# Autodesk Inventor assembly: ASY MSC 202 LEFT BOARD
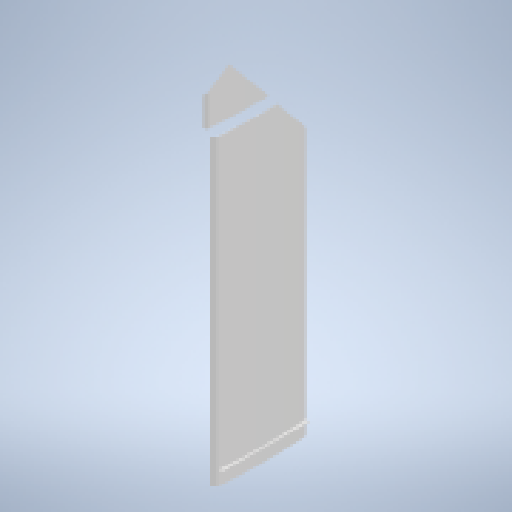
[picture p0: Inventor's stored thumbnail of the model, 512x512]
Saved by Autodesk Inventor 2025 (Build 290162010, 162A)
## iProperties
Created: 2024-07-21
Part Number: ASY MSC 202 LEFT BOARD
Document SubType Name: Assembly
Designer: pokla
Author: pokla
## Documents named in this file (6)
- C:\Users\admin\YandexDisk-badmisterfox\домашниий пк\Inventor\Manturovo\Manturovo_Se-clar\ASY MSC 202 LEFT BOARD.iam
- C:\Users\admin\YandexDisk-badmisterfox\домашниий пк\Inventor\Manturovo\Manturovo_Se-clar\MSC 052 rib board.ipt
- C:\Users\admin\YandexDisk-badmisterfox\домашниий пк\Inventor\Manturovo\Manturovo_Se-clar\MSC 024 sheet board main.ipt
- C:\Users\admin\YandexDisk-badmisterfox\домашниий пк\Inventor\Manturovo\Manturovo_Se-clar\MSC 023 sheet board.ipt
- C:\Users\admin\YandexDisk-badmisterfox\домашниий пк\Inventor\Manturovo\Manturovo_Se-clar\MSC 025 sheet board withers 1.ipt
- C:\Users\admin\YandexDisk-badmisterfox\домашниий пк\Inventor\Manturovo\Manturovo_Se-clar\MSC 027 sheet board face 1.ipt
## Components (9 placed, 5 different names)
1. MSC 052 rib board.ipt:3 — Flush:4, Mate:1, Flush:5, Tangent:1, Tangent:2, Angle:1
2. MSC 024 sheet board main.ipt:1 — Rigid:20, Rigid:21
3. MSC 024 sheet board main.ipt:2 — Rigid:21, Rigid:22
4. MSC 024 sheet board main.ipt:3 — Rigid:22, Rigid:23
5. MSC 024 sheet board main.ipt:4 — Rigid:23, Rigid:24
6. MSC 024 sheet board main.ipt:5 — Rigid:24, Rigid:25
7. MSC 023 sheet board.ipt:1 — Flush:4, Mate:2, Tangent:1, Tangent:2, Angle:1, Rigid:20
8. MSC 025 sheet board withers 1.ipt:1 — Rigid:25
9. MSC 027 sheet board face 1.ipt:1
## Relationships (13: WeldJoint 6, Flush 2, Mate 2, Tangent 2, Angle 1)
- Flush:4 (304 mm): MSC 052 rib board.ipt:3 ↔ MSC 023 sheet board.ipt:1
- Mate:1: MSC 052 rib board.ipt:3
- Flush:5: MSC 052 rib board.ipt:3
- Mate:2: MSC 023 sheet board.ipt:1
- Tangent:1: MSC 052 rib board.ipt:3 ↔ MSC 023 sheet board.ipt:1
- Tangent:2: MSC 052 rib board.ipt:3 ↔ MSC 023 sheet board.ipt:1
- Angle:1 (0 deg): MSC 052 rib board.ipt:3 ↔ MSC 023 sheet board.ipt:1
- Rigid:20 [WeldJoint]: MSC 024 sheet board main.ipt:1 ↔ MSC 023 sheet board.ipt:1
- Rigid:21 [WeldJoint]: MSC 024 sheet board main.ipt:1 ↔ MSC 024 sheet board main.ipt:2
- Rigid:22 [WeldJoint]: MSC 024 sheet board main.ipt:2 ↔ MSC 024 sheet board main.ipt:3
- Rigid:23 [WeldJoint]: MSC 024 sheet board main.ipt:3 ↔ MSC 024 sheet board main.ipt:4
- Rigid:24 [WeldJoint]: MSC 024 sheet board main.ipt:4 ↔ MSC 024 sheet board main.ipt:5
- Rigid:25 [WeldJoint]: MSC 024 sheet board main.ipt:5 ↔ MSC 025 sheet board withers 1.ipt:1
